# Autodesk Inventor assembly: Assembly1
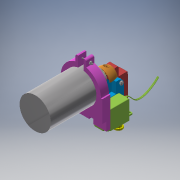
[picture p0: Inventor's stored thumbnail of the model, 180x180]
Saved by Autodesk Inventor 2016 (Build 200138000, 138)
## iProperties
Created: 2016-04-17
Part Number: Assembly1
Document SubType Name: Assembly
Designer: amenoni
Author: amenoni
## Documents named in this file (14)
- Z:\Desarrollo\WetMaths\wetMaths-Arduino\wetMaths\HwDesigns\Assembly1.iam
- Z:\Desarrollo\WetMaths\wetMaths-Arduino\wetMaths\HwDesigns\SprayCan.ipt
- Z:\Desarrollo\WetMaths\wetMaths-Arduino\wetMaths\HwDesigns\Clamp.ipt
- Z:\Desarrollo\WetMaths\wetMaths-Arduino\wetMaths\HwDesigns\CanNozzle.ipt
- Z:\Desarrollo\WetMaths\wetMaths-Arduino\wetMaths\HwDesigns\Futaba S3004.ipt
- \\psf\Home\Documents\Inventor\Content Center Files\R2016\en-US\AS 1427(05)\AS 1427 - M2.5 x 25(5) II.ipt
- \\psf\Home\Documents\Inventor\Content Center Files\R2016\en-US\AS 1112 (2)\AS 1112 - M2.5  Type 5.ipt
- Z:\Desarrollo\WetMaths\wetMaths-Arduino\wetMaths\HwDesigns\lever_support.ipt
- Z:\Desarrollo\WetMaths\wetMaths-Arduino\wetMaths\HwDesigns\Lever.ipt
- \\psf\Home\Documents\Inventor\Content Center Files\R2016\en-US\AS 1427(05)\AS 1427 - M3.5 x 35(5) II.ipt
- \\psf\Home\Documents\Inventor\Content Center Files\R2016\en-US\AS 1112 (2)\AS 1112 - M3.5  Type 10.ipt
- Z:\Desarrollo\WetMaths\wetMaths-Arduino\wetMaths\HwDesigns\big_servo_arm.ipt
- Z:\Desarrollo\WetMaths\wetMaths-Arduino\wetMaths\HwDesigns\Puller.ipt
- \\psf\Home\Documents\Inventor\Content Center Files\R2016\en-US\AS 1427(05)\AS 1427 - M2.5 x 16(5) II.ipt
## Components (15 placed, 13 different names)
1. SprayCan:1 — Mate:2, Mate:3, Rigid:1
2. Clamp:1 — Insert:1, Insert:2, Mate:4, Mate:5, Mate:6, Mate:8, Mate:9, Rigid:1, Mate:13, Mate:15
3. CanNozzle:1 — Mate:2, Mate:3
4. AS 1427 H - Metric M2.5 x 25:1 — Insert:1
5. AS 1112 (2) - Metric M2.5  Type 5:1 — Insert:2
6. lever_support:1 — Mate:4, Mate:6, Insert:4, Mate:12, Mate:14
7. lever_support:2 — Mate:5, Mate:8, Mate:9, Mate:10, Mate:11, Insert:3, Mate:14
8. Lever:1 — Mate:10, Mate:11, Mate:16, Mate:17, Mate:19
9. AS 1427 H - Metric M3.5 x 35:1 — Insert:3
10. AS 1112 (2) - Metric M3.5  Type 10:1 — Insert:4
11. Futaba S3004:1 — Mate:12, Mate:13, Mate:15, Rotational:1
12. big_servo_arm:1 — Rotational:1
13. Puller:1 — Mate:16, Mate:17, Insert:5
14. AS 1427 H - Metric M2.5 x 16:1 — Insert:5, Mate:18
15. AS 1112 (2) - Metric M2.5  Type 5:2 — Mate:18, Mate:19
## Relationships (24: Mate 17, Insert 5, WeldJoint 1, RevoluteJoint 1)
- Mate:2: SprayCan:1 ↔ CanNozzle:1
- Mate:3 (2.5 mm): SprayCan:1 ↔ CanNozzle:1
- Insert:1: Clamp:1 ↔ AS 1427 H - Metric M2.5 x 25:1
- Insert:2: Clamp:1 ↔ AS 1112 (2) - Metric M2.5  Type 5:1
- Mate:4: Clamp:1 ↔ lever_support:1
- Mate:5: Clamp:1 ↔ lever_support:2
- Mate:6: Clamp:1 ↔ lever_support:1
- Mate:8: Clamp:1 ↔ lever_support:2
- Mate:9: Clamp:1 ↔ lever_support:2
- Mate:10: lever_support:2 ↔ Lever:1
- Mate:11: lever_support:2 ↔ Lever:1
- Rigid:1 [WeldJoint]: SprayCan:1 ↔ Clamp:1
- Insert:3: lever_support:2 ↔ AS 1427 H - Metric M3.5 x 35:1
- Insert:4: lever_support:1 ↔ AS 1112 (2) - Metric M3.5  Type 10:1
- Mate:12: lever_support:1 ↔ Futaba S3004:1
- Mate:13: Clamp:1 ↔ Futaba S3004:1
- Mate:14 (15 mm): lever_support:1 ↔ lever_support:2
- Mate:15: Clamp:1 ↔ Futaba S3004:1
- Rotational:1 [RevoluteJoint]: Futaba S3004:1 ↔ big_servo_arm:1
- Mate:16: Lever:1 ↔ Puller:1
- Mate:17: Lever:1 ↔ Puller:1
- Insert:5: Puller:1 ↔ AS 1427 H - Metric M2.5 x 16:1
- Mate:18: AS 1427 H - Metric M2.5 x 16:1 ↔ AS 1112 (2) - Metric M2.5  Type 5:2
- Mate:19: Lever:1 ↔ AS 1112 (2) - Metric M2.5  Type 5:2
